# Autodesk Inventor assembly: LeQuad_brushless
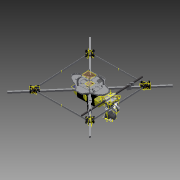
[picture p0: Inventor's stored thumbnail of the model, 180x180]
Saved by Autodesk Inventor 2015 SP1 (Build 190203100, 203)
## iProperties
Created: 2015-07-14
Part Number: LeQuad_brushless
Document SubType Name: Assembly
Designer: Alexandre Cherpillod
Author: Alexandre Cherpillod
## Documents named in this file (21)
- D:\_windows\_github_doc\MAVRIC\Mechanics\myCopter_CAD\Inventor\LeQuad_with_brushless.iam
- D:\_windows\_github_doc\MAVRIC\Mechanics\myCopter_CAD\Inventor\pcb_holder_gps_easy.ipt
- D:\_windows\_github_doc\MAVRIC\Mechanics\myCopter_CAD\Inventor\battery_holder_strong.ipt
- D:\_windows\_github_doc\MAVRIC\Mechanics\myCopter_CAD\Inventor\central_part_long.ipt
- D:\_windows\_github_doc\MAVRIC\Mechanics\myCopter_CAD\Inventor\carbon_stick.ipt
- D:\_windows\_github_doc\MAVRIC\Mechanics\myCopter_CAD\Inventor\support_motor_2_31mm.ipt
- D:\_windows\_github_doc\MAVRIC\Mechanics\myCopter_CAD\Inventor\support_motor_31mm.ipt
- D:\_windows\_github_doc\MAVRIC\Mechanics\myCopter_CAD\Inventor\carbon_blade.ipt
- D:\_windows\_github_doc\MAVRIC\Mechanics\myCopter_CAD\Inventor\battery_Zippy_Compact_3S_2200mAh_25C.ipt
- D:\_windows\_github_doc\MAVRIC\Mechanics\myCopter_CAD\Inventor\Gimbal_third_party\gimbal_stick_fixation.ipt
- D:\_windows\_github_doc\MAVRIC\Mechanics\myCopter_CAD\Inventor\Gimbal_third_party\gimbal_stick_fixation_big.ipt
- D:\_windows\_github_doc\MAVRIC\Mechanics\myCopter_CAD\Inventor\Gimbal_third_party\carbon_stick_gimbal.ipt
- D:\_windows\_github_doc\MAVRIC\Mechanics\myCopter_CAD\Inventor\Gimbal_third_party\carbon_tube_gimbal.ipt
- D:\_windows\_github_doc\MAVRIC\Mechanics\myCopter_CAD\Inventor\Gimbal_third_party\gimbal_fixation.ipt
- D:\_windows\_github_doc\MAVRIC\Mechanics\myCopter_CAD\Inventor\Gimbal_third_party\bump_black_small.ipt
- D:\_windows\_github_doc\MAVRIC\Mechanics\myCopter_CAD\Inventor\Misc\foot_holder.ipt
- D:\_windows\_github_doc\MAVRIC\Mechanics\myCopter_CAD\Inventor\Misc\foot_small.ipt
- D:\_windows\_github_doc\MAVRIC\Mechanics\myCopter_CAD\Inventor\Misc\foot_big.ipt
- D:\_windows\_github_doc\MAVRIC\Mechanics\myCopter_CAD\Inventor\Gimbal_Brushless\gimbal_brushless.iam
- D:\_windows\_github_doc\MAVRIC\Mechanics\myCopter_CAD\Inventor\Gimbal_third_party\holder_board_basecam_simpleBCG_32bit_tiny.ipt
- D:\_windows\_github_doc\MAVRIC\Mechanics\myCopter_CAD\Inventor\Gimbal_third_party\basecam_simpleBCG_32bit_tiny.ipt
## Components (30 placed, 20 different names)
1. pcb_holder_gps_easy:1 — Flush:2, Flush:3, Flush:4, Mate:1, Mate:2, Mate:3, Mate:11, Flush:16, Mate:20, Mate:21, Mate:22, Flush:20, Mate:60
2. battery_holder_strong:1 — Flush:2, Flush:3, Flush:4, Mate:23
3. central_part_long:1 — Mate:1, Mate:2, Mate:3, Mate:4, Flush:5, Flush:6, Mate:5, Mate:6, Mate:7
4. carbon_stick:1 — Mate:4, Flush:5, Mate:6, Mate:8, Flush:12, Mate:9, Flush:13, Mate:24, Mate:25, Mate:48, Mate:49, Mate:61, Mate:62, Flush:22
5. carbon_stick:2 — Flush:6, Mate:5, Mate:7, Flush:7, Flush:9, Flush:11, Flush:10, Mate:26, Mate:27, Mate:46, Mate:47
6. support_motor_2_31mm:1 — Flush:11, Flush:10, Mate:10, Mate:12, Flush:19
7. support_motor_2_31mm:2 — Flush:7, Flush:9, Mate:13, Flush:21, Mate:59
8. support_motor_31mm:1 — Mate:8, Flush:12, Flush:14
9. support_motor_31mm:2 — Mate:9, Flush:13, Flush:15, Mate:14, Mate:18, Mate:19
10. carbon_blade:1 — Mate:10, Flush:14, Mate:11, Mate:12
11. carbon_blade:3 — Flush:15, Mate:13, Mate:14, Flush:16
12. carbon_blade:4 — Mate:18, Mate:19, Mate:20, Flush:19
13. battery_Zippy_Compact_3S_2200mAh_25C:1 — Mate:21, Mate:22, Mate:23
14. gimbal_stick_fixation:2 — Mate:24, Mate:25, Mate:29
15. gimbal_stick_fixation_big:1 — Mate:26, Mate:27, Mate:28, Mate:30, Mate:31, Mate:32
16. carbon_stick_gimbal:1 — Mate:28, Mate:29, Mate:30, Mate:33, Mate:34
17. carbon_tube_gimbal:1 — Mate:31, Mate:32
18. gimbal_fixation:1 — Mate:33, Mate:34, Flush:20, Mate:35, Mate:36, Mate:37, Mate:38, Mate:39, Mate:40, Mate:41, Mate:42
19. bump_black_small:1 — Mate:35, Mate:36, Mate:56, Mate:57
20. bump_black_small:2 — Mate:37, Mate:38, Mate:58
21. bump_black_small:3 — Mate:39, Mate:40
22. bump_black_small:4 — Mate:41, Mate:42
23. foot_holder:1 — Mate:48, Mate:49, Mate:54, Mate:55
24. foot_holder:2 — Mate:46, Mate:47, Mate:52, Mate:53
25. foot_small:2 — Mate:52, Mate:53
26. foot_big:1 — Mate:54, Mate:55
27. gimbal_brushless:1 [sub-assembly] — Mate:56, Mate:57, Mate:58
28. carbon_blade:5 — Flush:21, Mate:59, Mate:60
29. holder_board_basecam_simpleBCG_32bit_tiny:1 — Mate:61, Mate:62, Flush:22, Mate:63, Mate:64, Mate:65, Mate:66
30. basecam_simpleBCG_32bit_tiny:1 — Mate:63, Mate:64, Mate:65, Mate:66
## Relationships (76: Mate 58, Flush 18)
- Flush:2: pcb_holder_gps_easy:1 ↔ battery_holder_strong:1
- Flush:3: pcb_holder_gps_easy:1 ↔ battery_holder_strong:1
- Flush:4: pcb_holder_gps_easy:1 ↔ battery_holder_strong:1
- Mate:1: pcb_holder_gps_easy:1 ↔ central_part_long:1
- Mate:2: pcb_holder_gps_easy:1 ↔ central_part_long:1
- Mate:3 (-2.5 mm): pcb_holder_gps_easy:1 ↔ central_part_long:1
- Mate:4: central_part_long:1 ↔ carbon_stick:1
- Flush:5: central_part_long:1 ↔ carbon_stick:1
- Flush:6: central_part_long:1 ↔ carbon_stick:2
- Mate:5: central_part_long:1 ↔ carbon_stick:2
- Mate:6: central_part_long:1 ↔ carbon_stick:1
- Mate:7: central_part_long:1 ↔ carbon_stick:2
- Flush:7: carbon_stick:2 ↔ support_motor_2_31mm:2
- Flush:9: carbon_stick:2 ↔ support_motor_2_31mm:2
- Flush:11: carbon_stick:2 ↔ support_motor_2_31mm:1
- Flush:10: carbon_stick:2 ↔ support_motor_2_31mm:1
- Mate:8: carbon_stick:1 ↔ support_motor_31mm:1
- Flush:12: carbon_stick:1 ↔ support_motor_31mm:1
- Mate:9: carbon_stick:1 ↔ support_motor_31mm:2
- Flush:13: carbon_stick:1 ↔ support_motor_31mm:2
- Mate:10: support_motor_2_31mm:1 ↔ carbon_blade:1
- Flush:14: support_motor_31mm:1 ↔ carbon_blade:1
- Mate:11: pcb_holder_gps_easy:1 ↔ carbon_blade:1
- Mate:12: support_motor_2_31mm:1 ↔ carbon_blade:1
- Flush:15: support_motor_31mm:2 ↔ carbon_blade:3
- Mate:13: support_motor_2_31mm:2 ↔ carbon_blade:3
- Mate:14: support_motor_31mm:2 ↔ carbon_blade:3
- Flush:16: pcb_holder_gps_easy:1 ↔ carbon_blade:3
- Mate:18: support_motor_31mm:2 ↔ carbon_blade:4
- Mate:19: support_motor_31mm:2 ↔ carbon_blade:4
- Mate:20: pcb_holder_gps_easy:1 ↔ carbon_blade:4
- Mate:21 (-1 mm): pcb_holder_gps_easy:1 ↔ battery_Zippy_Compact_3S_2200mAh_25C:1
- Mate:22: pcb_holder_gps_easy:1 ↔ battery_Zippy_Compact_3S_2200mAh_25C:1
- Mate:23 (4 mm): battery_holder_strong:1 ↔ battery_Zippy_Compact_3S_2200mAh_25C:1
- Flush:19: support_motor_2_31mm:1 ↔ carbon_blade:4
- Mate:24: carbon_stick:1 ↔ gimbal_stick_fixation:2
- Mate:25: carbon_stick:1 ↔ gimbal_stick_fixation:2
- Mate:26: carbon_stick:2 ↔ gimbal_stick_fixation_big:1
- Mate:27: carbon_stick:2 ↔ gimbal_stick_fixation_big:1
- Mate:28: gimbal_stick_fixation_big:1 ↔ carbon_stick_gimbal:1
- Mate:29: gimbal_stick_fixation:2 ↔ carbon_stick_gimbal:1
- Mate:30: gimbal_stick_fixation_big:1 ↔ carbon_stick_gimbal:1
- Mate:31: gimbal_stick_fixation_big:1 ↔ carbon_tube_gimbal:1
- Mate:32 (2 mm): gimbal_stick_fixation_big:1 ↔ carbon_tube_gimbal:1
- Mate:33: carbon_stick_gimbal:1 ↔ gimbal_fixation:1
- Mate:34: carbon_stick_gimbal:1 ↔ gimbal_fixation:1
- Flush:20: pcb_holder_gps_easy:1 ↔ gimbal_fixation:1
- Mate:35: gimbal_fixation:1 ↔ bump_black_small:1
- Mate:36: gimbal_fixation:1 ↔ bump_black_small:1
- Mate:37: gimbal_fixation:1 ↔ bump_black_small:2
- Mate:38: gimbal_fixation:1 ↔ bump_black_small:2
- Mate:39: gimbal_fixation:1 ↔ bump_black_small:3
- Mate:40: gimbal_fixation:1 ↔ bump_black_small:3
- Mate:41: gimbal_fixation:1 ↔ bump_black_small:4
- Mate:42: gimbal_fixation:1 ↔ bump_black_small:4
- Mate:46: carbon_stick:2 ↔ foot_holder:2
- Mate:47: carbon_stick:2 ↔ foot_holder:2
- Mate:48: carbon_stick:1 ↔ foot_holder:1
- Mate:49: carbon_stick:1 ↔ foot_holder:1
- Mate:52: foot_holder:2 ↔ foot_small:2
- Mate:53: foot_holder:2 ↔ foot_small:2
- Mate:54: foot_holder:1 ↔ foot_big:1
- Mate:55: foot_holder:1 ↔ foot_big:1
- Mate:56: bump_black_small:1 ↔ gimbal_brushless:1
- Mate:57: bump_black_small:1 ↔ gimbal_brushless:1
- Mate:58: bump_black_small:2 ↔ gimbal_brushless:1
- Flush:21: support_motor_2_31mm:2 ↔ carbon_blade:5
- Mate:59: support_motor_2_31mm:2 ↔ carbon_blade:5
- Mate:60: pcb_holder_gps_easy:1 ↔ carbon_blade:5
- Mate:61: carbon_stick:1 ↔ holder_board_basecam_simpleBCG_32bit_tiny:1
- Mate:62: carbon_stick:1 ↔ holder_board_basecam_simpleBCG_32bit_tiny:1
- Flush:22 (170 mm): carbon_stick:1 ↔ holder_board_basecam_simpleBCG_32bit_tiny:1
- Mate:63: holder_board_basecam_simpleBCG_32bit_tiny:1 ↔ basecam_simpleBCG_32bit_tiny:1
- Mate:64: holder_board_basecam_simpleBCG_32bit_tiny:1 ↔ basecam_simpleBCG_32bit_tiny:1
- Mate:65: holder_board_basecam_simpleBCG_32bit_tiny:1 ↔ basecam_simpleBCG_32bit_tiny:1
- Mate:66: holder_board_basecam_simpleBCG_32bit_tiny:1 ↔ basecam_simpleBCG_32bit_tiny:1
